# Autodesk Inventor assembly: czlon_4_zloz
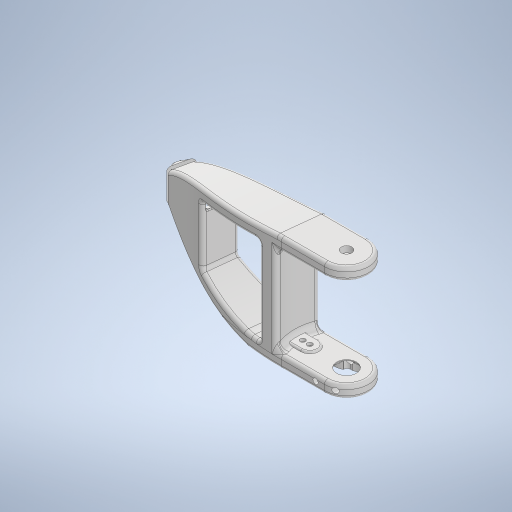
[picture p0: Inventor's stored thumbnail of the model, 512x512]
Saved by Autodesk Inventor 2023 (Build 270158000, 158)
## iProperties
Created: 2024-08-02
Part Number: czlon_4_zloz
Document SubType Name: Assembly
Designer: komputer
Author: komputer
## Documents named in this file (5)
- C:\Users\kamil\Documents\PROJECTS - repos\Robal-2.0\mechanics\czlon_4_zloz.iam
- C:\Users\kamil\Documents\PROJECTS - repos\Robal-2.0\mechanics\czlon4_pre_2.ipt
- C:\Users\kamil\Documents\PROJECTS - repos\Robal-2.0\mechanics\Micro Limit Switch\Micro Limit Switch.ipt
- C:\Users\kamil\Documents\PROJECTS - repos\Robal-2.0\mechanics\but.ipt
- C:\Users\kamil\Documents\PROJECTS - repos\Robal-2.0\mechanics\czlon4_pre_2_pokrywa.ipt
## Components (4 placed, 4 different names)
1. czlon4_pre_2:1 — Mate:1, Mate:2, Flush:1, Angle:1, Mate:3, Mate:4, Mate:5, Angle:2, Flush:2, Mate:6, Mate:7, Angle:3, Mate:8, Mate:9, Mate:10
2. but:1 — Flush:1, Angle:1, Mate:3, Mate:4
3. Micro Limit Switch:1 — Mate:5, Angle:2, Flush:2, Mate:6
4. czlon4_pre_2_pokrywa:1 — Mate:8, Mate:9, Mate:10
## Relationships (15: Mate 10, Angle 3, Flush 2)
- Mate:1: czlon4_pre_2:1
- Mate:2: czlon4_pre_2:1
- Flush:1: czlon4_pre_2:1 ↔ but:1
- Angle:1 (0 deg): czlon4_pre_2:1 ↔ but:1
- Mate:3 (0.5 mm): czlon4_pre_2:1 ↔ but:1
- Mate:4 (0.2 mm): czlon4_pre_2:1 ↔ but:1
- Mate:5: czlon4_pre_2:1 ↔ Micro Limit Switch:1
- Angle:2 (180 deg): czlon4_pre_2:1 ↔ Micro Limit Switch:1
- Flush:2: czlon4_pre_2:1 ↔ Micro Limit Switch:1
- Mate:6 (1.05 mm): czlon4_pre_2:1 ↔ Micro Limit Switch:1
- Mate:7: czlon4_pre_2:1
- Angle:3 (0 deg): czlon4_pre_2:1
- Mate:8: czlon4_pre_2:1 ↔ czlon4_pre_2_pokrywa:1
- Mate:9: czlon4_pre_2:1 ↔ czlon4_pre_2_pokrywa:1
- Mate:10: czlon4_pre_2:1 ↔ czlon4_pre_2_pokrywa:1
